# Autodesk Inventor assembly: Assembly1
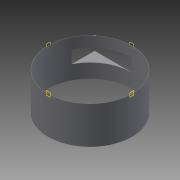
[picture p0: Inventor's stored thumbnail of the model, 180x180]
Saved by Autodesk Inventor 2018.2 (Build 222227000, 227)
## iProperties
Created: 2018-02-07
Part Number: Assembly1
Document SubType Name: Assembly
Designer: Rus
Author: Rus
## Documents named in this file (3)
- E:\Libraries\3D Objects\Central Vac Cyclone\V0_0\Assembly1.iam
- E:\Libraries\3D Objects\Central Vac Cyclone\V0_0\Cyclone Inlet.ipt
- E:\Libraries\3D Objects\Central Vac Cyclone\V0_0\Cyclone Main Straight Metal.ipt
## Components (3 placed, 3 different names)
1. Cyclone Main Inlet:1 — Flush:1
2. Cyclone Main Straight Metal:1 — Flush:1, Tangent:1, Mate:1, Mate:2
3. Cyclone Inlet:2 — Tangent:1, Mate:1, Mate:2
## Relationships (4: Mate 2, Flush 1, Tangent 1)
- Flush:1: Cyclone Main Inlet:1 ↔ Cyclone Main Straight Metal:1
- Tangent:1: Cyclone Main Straight Metal:1 ↔ Cyclone Inlet:2
- Mate:1: Cyclone Main Straight Metal:1 ↔ Cyclone Inlet:2
- Mate:2: Cyclone Main Straight Metal:1 ↔ Cyclone Inlet:2
